# Autodesk Inventor assembly: Sample 1
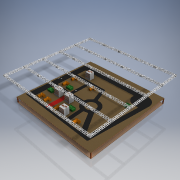
[picture p0: Inventor's stored thumbnail of the model, 180x180]
Saved by Autodesk Inventor 2019 (Build 230136000, 136)
## iProperties
Created: 2020-04-28
Part Number: Sample 1
Document SubType Name: Assembly
Designer: infinity
Author: infinity
## Documents named in this file (9)
- C:\Users\close\Desktop\BARC-ROAR\barc_hardware\Track Sample 2\Sample 2.iam
- C:\Users\close\Desktop\BARC-ROAR\barc_hardware\Track Sample 2\2ft stand.ipt
- C:\Users\close\Desktop\BARC-ROAR\barc_hardware\Track Sample 2\floor_50_50.ipt
- C:\Users\close\Desktop\BARC-ROAR\barc_hardware\Track Sample 2\Mcity track.ipt
- C:\Users\close\Desktop\BARC-ROAR\barc_hardware\Track Sample 2\house_1.ipt
- C:\Users\close\Desktop\BARC-ROAR\barc_hardware\Track Sample 2\apartment_1.ipt
- C:\Users\close\Desktop\BARC-ROAR\barc_hardware\Track Sample 2\building_1.ipt
- C:\Users\close\Desktop\BARC-ROAR\barc_hardware\Track Sample 2\car110th.ipt
- C:\Users\close\Desktop\BARC-ROAR\barc_hardware\Dependencies\truss rails\50ft.iam
## Components (24 placed, 8 different names)
1. 2ft stand:1 — Flush:45, Flush:46, Mate:57, Mate:58, Flush:47, Flush:48
2. floor_50_50:1 — Flush:45, Flush:46, Mate:57, Mate:60
3. Mcity track:1 — Mate:58, Flush:47, Flush:48, Flush:55, Flush:59, Flush:63, Tangent:1, Tangent:2, Tangent:3, Tangent:4, Tangent:5, Tangent:6
4. house_1:1 — Flush:50, Flush:51
5. house_1:2 — Flush:51, Flush:52
6. house_1:3 — Flush:53
7. house_1:4 — Flush:52, Flush:54, Flush:55
8. house_1:5 — Flush:49, Flush:50
9. house_1:6 — Flush:53, Flush:54
10. house_1:7 — Flush:49
11. apartment_1:1 — Flush:56
12. apartment_1:2 — Flush:56, Flush:57
13. apartment_1:3 — Flush:57, Flush:58
14. apartment_1:4 — Flush:58, Flush:59
15. building_1:1 — Flush:60, Flush:61
16. building_1:2 — Flush:60, Flush:62
17. building_1:3 — Flush:61, Flush:63
18. building_1:4 — Flush:62
19. car110th:1 — Tangent:3, Tangent:4
20. car110th:2 — Tangent:2, Tangent:6
21. car110th:3 — Tangent:1, Tangent:5
22. car110th:4
23. car110th:5
24. 50ft:1 [sub-assembly] — Mate:59
## Relationships (30: Flush 20, Tangent 6, Mate 4)
- Flush:45: 2ft stand:1 ↔ floor_50_50:1
- Flush:46: 2ft stand:1 ↔ floor_50_50:1
- Mate:57: 2ft stand:1 ↔ floor_50_50:1
- Mate:58: 2ft stand:1 ↔ Mcity track:1
- Flush:47: 2ft stand:1 ↔ Mcity track:1
- Flush:48: 2ft stand:1 ↔ Mcity track:1
- Flush:49: house_1:5 ↔ house_1:7
- Flush:50: house_1:1 ↔ house_1:5
- Flush:51: house_1:1 ↔ house_1:2
- Flush:52: house_1:2 ↔ house_1:4
- Flush:53: house_1:3 ↔ house_1:6
- Flush:54: house_1:4 ↔ house_1:6
- Flush:55: Mcity track:1 ↔ house_1:4
- Flush:56: apartment_1:1 ↔ apartment_1:2
- Flush:57: apartment_1:2 ↔ apartment_1:3
- Flush:58: apartment_1:3 ↔ apartment_1:4
- Flush:59: Mcity track:1 ↔ apartment_1:4
- Flush:60: building_1:1 ↔ building_1:2
- Flush:61: building_1:1 ↔ building_1:3
- Flush:62: building_1:2 ↔ building_1:4
- Flush:63: Mcity track:1 ↔ building_1:3
- Tangent:1: Mcity track:1 ↔ car110th:3
- Tangent:2: Mcity track:1 ↔ car110th:2
- Tangent:3: Mcity track:1 ↔ car110th:1
- Tangent:4: Mcity track:1 ↔ car110th:1
- Tangent:5: Mcity track:1 ↔ car110th:3
- Tangent:6: Mcity track:1 ↔ car110th:2
- Flush:64 (4572 mm)
- Mate:59: 50ft:1
- Mate:60: floor_50_50:1
